# Autodesk Inventor assembly: 61300711121 (rev1)
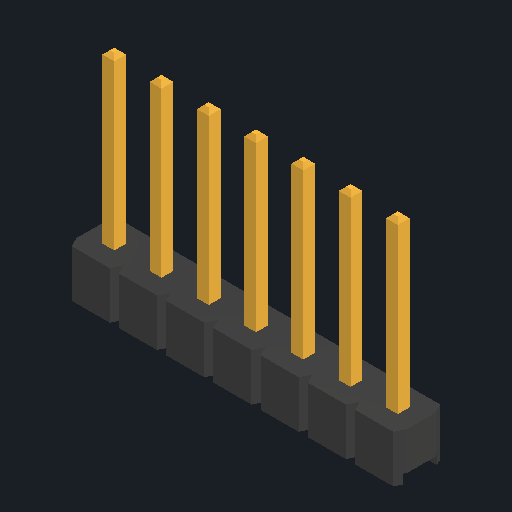
[picture p0: Inventor's stored thumbnail of the model, 512x512]
Saved by Autodesk Inventor 2022 (Build 260153000, 153)
## iProperties
Company: Unknown
Created: 2021-04-15
Part Number: 61300711121 (rev1)
Description: Unknown
Document SubType Name: Assembly
Designer: dvorakj
Authority: Unknown
Sending System: Solid Edge
Preprocessor: ST-DEVELOPER v16.7
Title: 61300711121
Author: Unknown
## Documents named in this file (3)
- C:\Users\dvorakj\Documents\Inventor\Bakalarka\MS5607\Pin header\61300711121 (rev1)plastic on top.iam
- C:\Users\dvorakj\Documents\Inventor\Bakalarka\MS5607\Pin header\61300711121.ipt
- C:\Users\dvorakj\Documents\Inventor\Bakalarka\MS5607\Pin header\6130xx11121_PIN.ipt
## Components (8 placed, 2 different names)
1. 61300711121 — Flush:1
2. 6130xx11121_PIN
3. 6130xx11121_PIN:1
4. 6130xx11121_PIN:2
5. 6130xx11121_PIN:3
6. 6130xx11121_PIN:4
7. 6130xx11121_PIN:5
8. 6130xx11121_PIN:6 — Flush:1
## Relationships (1: Flush 1)
- Flush:1: 61300711121 ↔ 6130xx11121_PIN:6
